# Autodesk Inventor assembly: Zespół1
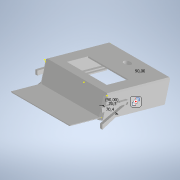
[picture p0: Inventor's stored thumbnail of the model, 180x180]
Saved by Autodesk Inventor 2020 (Build 240168000, 168)
## iProperties
Created: 2019-11-16
Part Number: Zespół1
Document SubType Name: Assembly
Designer: Hubert Słomion
Author: Hubert Słomion
## Documents named in this file (5)
- C:\Users\Hubert Słomion\Desktop\studia\inzynierka\fotobudka_cad\Zespół1.iam
- C:\Users\Hubert Słomion\Desktop\studia\inzynierka\fotobudka_cad\Część1.ipt
- C:\Users\Hubert Słomion\Desktop\studia\inzynierka\fotobudka_cad\klapa.ipt
- C:\Users\Hubert Słomion\Desktop\studia\inzynierka\fotobudka_cad\wiatrak.ipt
- C:\Users\Hubert Słomion\Desktop\studia\inzynierka\fotobudka_cad\stojak.ipt
## Components (5 placed, 4 different names)
1. Część1:1 — Zestawiające:1, Zestawiające:2, Zestawiające:4, Zestawiające:5, Równoległe:1, Zestawiające:6, Zestawiające:7, Zestawiające:8, Zestawiające:9
2. klapa:1 — Zestawiające:1, Zestawiające:2
3. wiatrak:1 — Zestawiające:4, Zestawiające:5
4. stojak:1 — Zestawiające:6, Zestawiające:7, Równoległe:2
5. stojak:2 — Zestawiające:8, Zestawiające:9, Równoległe:2
## Relationships (10: Mate 8, Flush 2)
- Zestawiające:1 [Mate]: Część1:1 ↔ klapa:1
- Zestawiające:2 [Mate]: Część1:1 ↔ klapa:1
- Zestawiające:4 [Mate]: Część1:1 ↔ wiatrak:1
- Zestawiające:5 [Mate]: Część1:1 ↔ wiatrak:1
- Równoległe:1 [Flush] (-175.5 mm): Część1:1
- Zestawiające:6 [Mate]: Część1:1 ↔ stojak:1
- Zestawiające:7 [Mate]: Część1:1 ↔ stojak:1
- Zestawiające:8 [Mate]: Część1:1 ↔ stojak:2
- Zestawiające:9 [Mate]: Część1:1 ↔ stojak:2
- Równoległe:2 [Flush]: stojak:1 ↔ stojak:2
